# Autodesk Inventor assembly: MECANISMO DE COMPACTADO
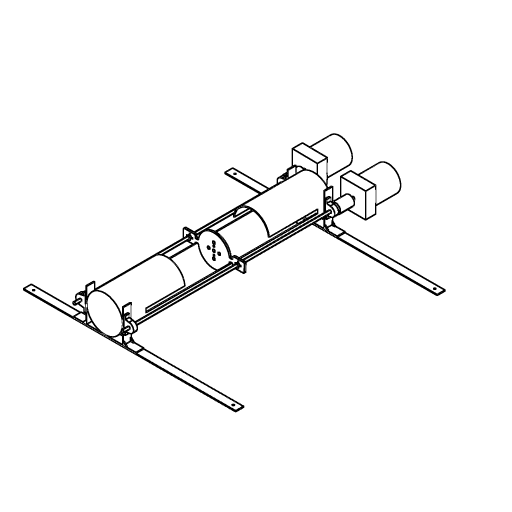
[picture p0: Inventor's stored thumbnail of the model, 512x512]
Saved by Autodesk Inventor 2024 (Build 280153000, 153)
## iProperties
Created: 2024-05-26
Part Number: MECANISMO DE COMPACTADO
Document SubType Name: Assembly
Designer: Jhuliams
Author: Jhuliams
## Documents named in this file (10)
- C:\Users\Jhuliams\Documents\GitHub\RECICLADOR_MODELO_3D\MECANISMO DE COMPACTADO\MECANISMO DE COMPACTADO.iam
- C:\Users\Jhuliams\Documents\GitHub\RECICLADOR_MODELO_3D\MECANISMO DE COMPACTADO\GUIA_DE_OBJETO.ipt
- C:\Users\Jhuliams\Documents\GitHub\RECICLADOR_MODELO_3D\MECANISMO DE COMPACTADO\TAPA QUE DESPLAZA CON TORNILLOS.ipt
- C:\Users\Jhuliams\Documents\GitHub\RECICLADOR_MODELO_3D\MECANISMO DE COMPACTADO\TUERCA DE HUSILLO.ipt
- C:\Users\Jhuliams\Documents\GitHub\RECICLADOR_MODELO_3D\MECANISMO DE COMPACTADO\TORNILLO DEPOTENCIA.ipt
- C:\Users\Jhuliams\Documents\GitHub\RECICLADOR_MODELO_3D\MECANISMO DE COMPACTADO\SOPORTE DE GUIA.ipt
- C:\Users\Jhuliams\Documents\GitHub\RECICLADOR_MODELO_3D\MECANISMO DE COMPACTADO\ACOPLE HELICOIDAL.ipt
- C:\Users\Jhuliams\Documents\GitHub\RECICLADOR_MODELO_3D\MECANISMO DE COMPACTADO\MOTOR DC.ipt
- C:\Users\Jhuliams\Documents\GitHub\RECICLADOR_MODELO_3D\MECANISMO DE COMPACTADO\RODAMIENTO DE TORNILLO.ipt
- C:\Users\Jhuliams\Documents\GitHub\RECICLADOR_MODELO_3D\MECANISMO DE COMPACTADO\PLETINA PARA GUIA CILINDRICA.ipt
## Components (18 placed, 9 different names)
1. PLETINA PARA GUIA CILINDRICA:1 — Mate:1, Flush:3
2. PLETINA PARA GUIA CILINDRICA:2 — Flush:4
3. SOPORTE DE GUIA:1 — Flush:1, Flush:2, Flush:4, Flush:9, Flush:10
4. SOPORTE DE GUIA:2 — Flush:1, Flush:2, Mate:1, Flush:3, Flush:5, Tangent:1, Tangent:2, Flush:6, Flush:7, Flush:8
5. GUIA_DE_OBJETO:1 — Flush:5, Tangent:1, Tangent:2, Mate:6, Mate:7, Mate:8, Flush:6
6. TORNILLO DEPOTENCIA:1 — Mate:9, Mate:13, Mate:14, Mate:16, Mate:22
7. TORNILLO DEPOTENCIA:2 — Mate:10, Mate:11, Mate:12, Mate:15, Mate:21
8. TAPA QUE DESPLAZA CON TORNILLOS:1 — Mate:6, Mate:7, Mate:8, Mate:9, Mate:10, Mate:17, Mate:18, Mate:19, Mate:20
9. RODAMIENTO DE TORNILLO:1 — Mate:14, Flush:7
10. RODAMIENTO DE TORNILLO:2 — Mate:13, Flush:9, Mate:23
11. RODAMIENTO DE TORNILLO:3 — Mate:11, Flush:8
12. RODAMIENTO DE TORNILLO:4 — Mate:12, Flush:10, Mate:24
13. TUERCA DE HUSILLO:1 — Mate:16, Mate:17, Mate:20
14. TUERCA DE HUSILLO:2 — Mate:15, Mate:18, Mate:19
15. ACOPLE HELICOIDAL:1 — Mate:22, Mate:23, Mate:26, Mate:28
16. ACOPLE HELICOIDAL:2 — Mate:21, Mate:24, Mate:25, Mate:27
17. MOTOR DC:1 — Mate:25, Mate:27
18. MOTOR DC:2 — Mate:26, Mate:28
## Relationships (36: Mate 24, Flush 10, Tangent 2)
- Flush:1: SOPORTE DE GUIA:1 ↔ SOPORTE DE GUIA:2
- Flush:2: SOPORTE DE GUIA:1 ↔ SOPORTE DE GUIA:2
- Mate:1: PLETINA PARA GUIA CILINDRICA:1 ↔ SOPORTE DE GUIA:2
- Flush:3: PLETINA PARA GUIA CILINDRICA:1 ↔ SOPORTE DE GUIA:2
- Flush:4: PLETINA PARA GUIA CILINDRICA:2 ↔ SOPORTE DE GUIA:1
- Flush:5: SOPORTE DE GUIA:2 ↔ GUIA_DE_OBJETO:1
- Tangent:1: SOPORTE DE GUIA:2 ↔ GUIA_DE_OBJETO:1
- Tangent:2: SOPORTE DE GUIA:2 ↔ GUIA_DE_OBJETO:1
- Mate:6: GUIA_DE_OBJETO:1 ↔ TAPA QUE DESPLAZA CON TORNILLOS:1
- Mate:7 (1 mm): GUIA_DE_OBJETO:1 ↔ TAPA QUE DESPLAZA CON TORNILLOS:1
- Mate:8 (1 mm): GUIA_DE_OBJETO:1 ↔ TAPA QUE DESPLAZA CON TORNILLOS:1
- Mate:9: TORNILLO DEPOTENCIA:1 ↔ TAPA QUE DESPLAZA CON TORNILLOS:1
- Mate:10: TORNILLO DEPOTENCIA:2 ↔ TAPA QUE DESPLAZA CON TORNILLOS:1
- Flush:6 (-51.5 mm): SOPORTE DE GUIA:2 ↔ GUIA_DE_OBJETO:1
- Mate:11: TORNILLO DEPOTENCIA:2 ↔ RODAMIENTO DE TORNILLO:3
- Mate:12: TORNILLO DEPOTENCIA:2 ↔ RODAMIENTO DE TORNILLO:4
- Mate:13: TORNILLO DEPOTENCIA:1 ↔ RODAMIENTO DE TORNILLO:2
- Mate:14: TORNILLO DEPOTENCIA:1 ↔ RODAMIENTO DE TORNILLO:1
- Flush:7: SOPORTE DE GUIA:2 ↔ RODAMIENTO DE TORNILLO:1
- Flush:8: SOPORTE DE GUIA:2 ↔ RODAMIENTO DE TORNILLO:3
- Flush:9: SOPORTE DE GUIA:1 ↔ RODAMIENTO DE TORNILLO:2
- Flush:10: SOPORTE DE GUIA:1 ↔ RODAMIENTO DE TORNILLO:4
- Mate:15: TORNILLO DEPOTENCIA:2 ↔ TUERCA DE HUSILLO:2
- Mate:16: TORNILLO DEPOTENCIA:1 ↔ TUERCA DE HUSILLO:1
- Mate:17: TAPA QUE DESPLAZA CON TORNILLOS:1 ↔ TUERCA DE HUSILLO:1
- Mate:18: TAPA QUE DESPLAZA CON TORNILLOS:1 ↔ TUERCA DE HUSILLO:2
- Mate:19: TAPA QUE DESPLAZA CON TORNILLOS:1 ↔ TUERCA DE HUSILLO:2
- Mate:20: TAPA QUE DESPLAZA CON TORNILLOS:1 ↔ TUERCA DE HUSILLO:1
- Mate:21: TORNILLO DEPOTENCIA:2 ↔ ACOPLE HELICOIDAL:2
- Mate:22: TORNILLO DEPOTENCIA:1 ↔ ACOPLE HELICOIDAL:1
- Mate:23 (5 mm): RODAMIENTO DE TORNILLO:2 ↔ ACOPLE HELICOIDAL:1
- Mate:24 (5 mm): RODAMIENTO DE TORNILLO:4 ↔ ACOPLE HELICOIDAL:2
- Mate:25: ACOPLE HELICOIDAL:2 ↔ MOTOR DC:1
- Mate:26: ACOPLE HELICOIDAL:1 ↔ MOTOR DC:2
- Mate:27 (12 mm): ACOPLE HELICOIDAL:2 ↔ MOTOR DC:1
- Mate:28 (12 mm): ACOPLE HELICOIDAL:1 ↔ MOTOR DC:2
